# Autodesk Inventor assembly: Wing Right
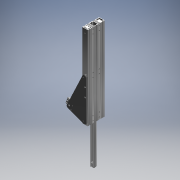
[picture p0: Inventor's stored thumbnail of the model, 180x180]
Saved by Autodesk Inventor 2019 (Build 230136000, 136)
## iProperties
Part Number: Wing Right
Document SubType Name: Assembly
Designer: Delta
Author: Delta
## Documents named in this file (5)
- C:\Robotics\CAD\2019-20_CAD\Collection\Wing Right.iam
- C:\Robotics\CAD\2019-20_CAD\Collection\Triangle axle slide connector.ipt
- C:\Robotics\CAD\COTSParts\Rev\REV-41-1683 Bear Blocks.ipt
- C:\Robotics\CAD\COTSParts\Misumi_Slides\AIS2018\SAR330.iam
- C:\Robotics\CAD\2018-19_CAD\2019-20_CAD\offseason\slide conector.ipt
## Components (7 placed, 4 different names)
1. Triangle axle slide connector:1 — Mate:3, Angle:1, Mate:6, Mate:8, Angle:2, Mate:21
2. REV-41-1683 Bear Blocks:1 — Mate:3, Angle:1, Mate:6
3. SAR330:1 [sub-assembly] — Mate:8, Angle:2, Mate:9, Mate:10, Mate:11, Mate:21
4. SAR330:2 [sub-assembly] — Mate:12, Mate:13, Mate:14, Mate:15, Mate:16, Mate:17
5. slide conector:1 — Mate:9, Mate:10, Mate:11, Mate:12, Mate:13, Mate:14
6. slide conector:2 — Mate:15, Mate:16, Mate:17, Mate:18, Mate:19, Mate:20
7. SAR330:3 [sub-assembly] — Mate:18, Mate:19, Mate:20
## Relationships (18: Mate 16, Angle 2)
- Mate:3: Triangle axle slide connector:1 ↔ REV-41-1683 Bear Blocks:1
- Angle:1 (0 deg): Triangle axle slide connector:1 ↔ REV-41-1683 Bear Blocks:1
- Mate:6: Triangle axle slide connector:1 ↔ REV-41-1683 Bear Blocks:1
- Mate:8: Triangle axle slide connector:1 ↔ SAR330:1
- Angle:2 (0 deg): Triangle axle slide connector:1 ↔ SAR330:1
- Mate:9: SAR330:1 ↔ slide conector:1
- Mate:10: SAR330:1 ↔ slide conector:1
- Mate:11: SAR330:1 ↔ slide conector:1
- Mate:12: SAR330:2 ↔ slide conector:1
- Mate:13: SAR330:2 ↔ slide conector:1
- Mate:14: SAR330:2 ↔ slide conector:1
- Mate:15: SAR330:2 ↔ slide conector:2
- Mate:16: SAR330:2 ↔ slide conector:2
- Mate:17: SAR330:2 ↔ slide conector:2
- Mate:18: slide conector:2 ↔ SAR330:3
- Mate:19: slide conector:2 ↔ SAR330:3
- Mate:20: slide conector:2 ↔ SAR330:3
- Mate:21: Triangle axle slide connector:1 ↔ SAR330:1
